# Autodesk Inventor assembly: Assembly2
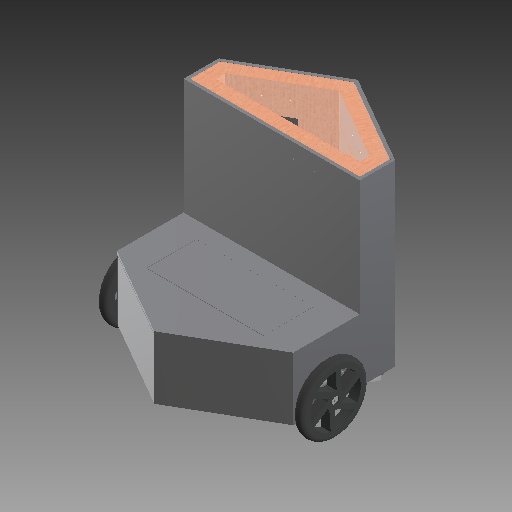
[picture p0: Inventor's stored thumbnail of the model, 512x512]
Saved by Autodesk Inventor 2017 (Build 210142000, 142)
## iProperties
Created: 2018-10-17
Part Number: Assembly2
Document SubType Name: Assembly
Designer: Administrator
Author: Administrator
## Documents named in this file (5)
- C:\Users\Dell\Documents\GitHub\tr2\Base\Base.iam
- C:\Users\Dell\Documents\GitHub\tr2\Base\Base Cover Assembly.iam
- C:\Users\Dell\Documents\GitHub\tr2\Base\Base Chassis Assembly.iam
- C:\Users\Dell\Documents\GitHub\tr2\Wheel Assembly\Wheel Assembly, Right.iam
- C:\Users\Dell\Documents\GitHub\tr2\Base\Caster Wheel\004. Castor Wheel Full_TOP.iam
## Components (6 placed, 4 different names)
1. Base Cover Assembly:1 [sub-assembly] — Mate:132, Mate:133, Mate:134
2. Base Chassis Assembly:1 [sub-assembly] — Mate:121, Mate:123, Flush:3, Mate:127, Flush:4, Flush:5, Mate:128, Mate:130, Mate:131, Mate:132, Mate:133, Mate:134, Mate:135, Mate:136, Flush:6, Flush:7, Mate:137, Mate:138
3. Wheel Assembly, Right:1 [sub-assembly] — Flush:5, Mate:128, Mate:130
4. Wheel Assembly, Right:2 [sub-assembly] — Mate:127, Flush:4, Mate:131
5. 004. Castor Wheel Full_TOP:1 [sub-assembly] — Mate:135, Flush:7, Mate:137
6. 004. Castor Wheel Full_TOP:2 [sub-assembly] — Mate:136, Flush:6, Mate:138
## Relationships (18: Mate 13, Flush 5)
- Mate:121: Base Chassis Assembly:1
- Mate:123: Base Chassis Assembly:1
- Flush:3: Base Chassis Assembly:1
- Mate:127: Base Chassis Assembly:1 ↔ Wheel Assembly, Right:2
- Flush:4: Base Chassis Assembly:1 ↔ Wheel Assembly, Right:2
- Flush:5: Base Chassis Assembly:1 ↔ Wheel Assembly, Right:1
- Mate:128: Base Chassis Assembly:1 ↔ Wheel Assembly, Right:1
- Mate:130: Base Chassis Assembly:1 ↔ Wheel Assembly, Right:1
- Mate:131: Base Chassis Assembly:1 ↔ Wheel Assembly, Right:2
- Mate:132: Base Cover Assembly:1 ↔ Base Chassis Assembly:1
- Mate:133: Base Cover Assembly:1 ↔ Base Chassis Assembly:1
- Mate:134: Base Cover Assembly:1 ↔ Base Chassis Assembly:1
- Mate:135: Base Chassis Assembly:1 ↔ 004. Castor Wheel Full_TOP:1
- Mate:136: Base Chassis Assembly:1 ↔ 004. Castor Wheel Full_TOP:2
- Flush:6: Base Chassis Assembly:1 ↔ 004. Castor Wheel Full_TOP:2
- Flush:7: Base Chassis Assembly:1 ↔ 004. Castor Wheel Full_TOP:1
- Mate:137: Base Chassis Assembly:1 ↔ 004. Castor Wheel Full_TOP:1
- Mate:138: Base Chassis Assembly:1 ↔ 004. Castor Wheel Full_TOP:2
